# Autodesk Inventor assembly: LidAndFeeder
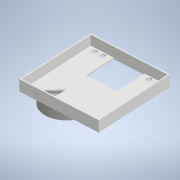
[picture p0: Inventor's stored thumbnail of the model, 180x180]
Saved by Autodesk Inventor 2020 (Build 240168000, 168)
## iProperties
Created: 2020-04-03
Part Number: LidAndFeeder
Document SubType Name: Assembly
Designer: jared.jones280
Author: jared.jones280
## Documents named in this file (3)
- H:\Autodesk\LidAndFeeder.iam
- \\toaster\homes\j\a\jared.jones280\nt\Autodesk\FixedLid.ipt
- \\toaster\homes\j\a\jared.jones280\nt\Autodesk\WheelFeeder.iam
## Components (2 placed, 2 different names)
1. FixedLid:1 — Mate:1, Flush:1, Flush:2
2. WheelFeeder:1 [sub-assembly] — Mate:1, Flush:1, Flush:2
## Relationships (3: Flush 2, Mate 1)
- Mate:1: FixedLid:1 ↔ WheelFeeder:1
- Flush:1: FixedLid:1 ↔ WheelFeeder:1
- Flush:2: FixedLid:1 ↔ WheelFeeder:1
